# Autodesk Inventor assembly: UmlenkrolleHalterDoppelt
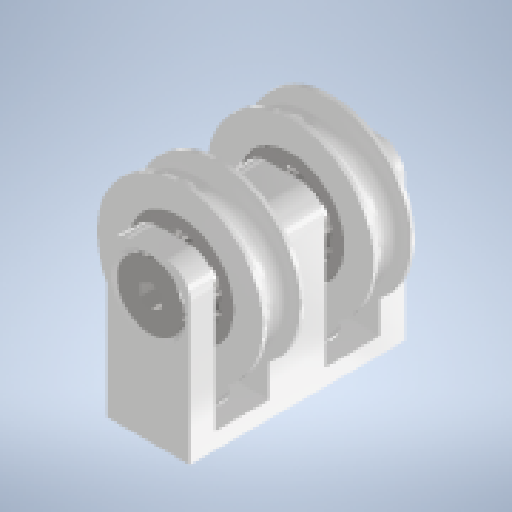
[picture p0: Inventor's stored thumbnail of the model, 512x512]
Saved by Autodesk Inventor 2025 (Build 290162010, 162A)
## iProperties
Created: 2024-11-19
Part Number: UmlenkrolleHalterDoppelt
Document SubType Name: Assembly
Designer: Admin
Mass: 13.6278 g
Surface Area: 66.014 cm^2
Volume: 4.89201 cm^3
Density: 2.78572 g/cm^3
Author: Admin
## Documents named in this file (5)
- C:\Users\Admin\Documents\Inventor\Krandemonstrator\UmlenkrolleHalterDoppelt.iam
- C:\Users\Admin\Documents\Inventor\Krandemonstrator\Umlenkrolle.iam
- C:\Users\Admin\Documents\Inventor\Content Center Files\R2025\de-DE\AS 1237 (2.1)\AS 1237 - 4.ipt
- C:\Users\Admin\Documents\Inventor\Krandemonstrator\HalterUmlenkrolleDPL.ipt
- C:\Users\Admin\Documents\Inventor\Content Center Files\R2025\de-DE\DIN 7991(2)\DIN 7991 - M4x25.ipt
## Components (8 placed, 4 different names)
1. Umlenkrolle:1 [sub-assembly] — Drehbar:1, Drehbar:2
2. AS 1237 (2.1) 4:1 — Starr:3, Drehbar:3
3. AS 1237 (2.1) 4:2 — Drehbar:2
4. HalterUmlenkrolleDPL:1 — Starr:1, Starr:2, Starr:3
5. AS 1237 (2.1) 4:3 — Starr:2, Drehbar:1
6. DIN 7991 M4x25:1 — Starr:1
7. Umlenkrolle:2 [sub-assembly] — Drehbar:3, Drehbar:4
8. AS 1237 (2.1) 4:4 — Drehbar:4
## Relationships (7: RevoluteJoint 4, WeldJoint 3)
- Starr:1 [WeldJoint]: HalterUmlenkrolleDPL:1 ↔ DIN 7991 M4x25:1
- Starr:2 [WeldJoint]: HalterUmlenkrolleDPL:1 ↔ AS 1237 (2.1) 4:3
- Starr:3 [WeldJoint]: AS 1237 (2.1) 4:1 ↔ HalterUmlenkrolleDPL:1
- Drehbar:1 [RevoluteJoint]: Umlenkrolle:1 ↔ AS 1237 (2.1) 4:3
- Drehbar:2 [RevoluteJoint]: Umlenkrolle:1 ↔ AS 1237 (2.1) 4:2
- Drehbar:3 [RevoluteJoint]: AS 1237 (2.1) 4:1 ↔ Umlenkrolle:2
- Drehbar:4 [RevoluteJoint]: Umlenkrolle:2 ↔ AS 1237 (2.1) 4:4
